# Autodesk Inventor assembly: main_assembly
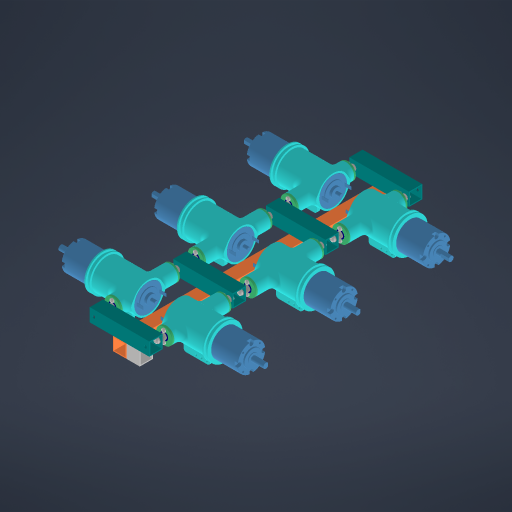
[picture p0: Inventor's stored thumbnail of the model, 512x512]
Saved by Autodesk Inventor 2024 (Build 280153000, 153)
## iProperties
Created: 2023-04-13
Part Number: main_assembly
Document SubType Name: Assembly
Designer: user
Author: user
## Documents named in this file (2)
- D:\DOC\Robot\3d\main_assembly.iam
- D:\DOC\Robot\3d\base\base_assembly.iam
## Components (1 placed, 1 different names)
1. base_assembly:1 [sub-assembly] — Совмещение:1, Совмещение:2, Совмещение:3, Совмещение:4
## Relationships (4: Mate 4)
- Совмещение:1 [Mate]: base_assembly:1
- Совмещение:2 [Mate]: base_assembly:1
- Совмещение:3 [Mate]: base_assembly:1
- Совмещение:4 [Mate]: base_assembly:1
